# Autodesk Inventor assembly: Trappe Haute
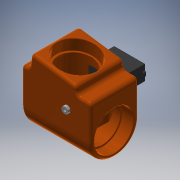
[picture p0: Inventor's stored thumbnail of the model, 180x180]
Saved by Autodesk Inventor 2016 SP1 (Build 200210100, 210)
## iProperties
Created: 2017-04-27
Part Number: Trappe Haute
Material: Générique
Document SubType Name: Assembly
Designer: dimercur
Author: dimercur
## Documents named in this file (6)
- D:\Users\dimercur\Documents\git\dev-gei\dev-gei2\Circuit-a-Bille\Trappe Haute.iam
- D:\Users\dimercur\Documents\git\dev-gei\dev-gei2\Circuit-a-Bille\Trappe Haute.ipt
- D:\Users\dimercur\Documents\git\dev-gei\dev-gei2\Circuit-a-Bille\Loquet Haut.ipt
- D:\Users\dimercur\Documents\git\dev-gei\dev-gei2\Circuit-a-Bille\Pieces importées\Futaba-s3004.ipt
- D:\Users\dimercur\Documents\Inventor\Content Center Files\R2016\fr-FR\NF E 25-130\NF E 25-130 - M5 x 10.ipt
- D:\Users\dimercur\Documents\Inventor\Content Center Files\R2016\fr-FR\ISO 7049 - F-H(2)\ISO 7049 - ST 3,5 x 9,5 - F - H.ipt
## Components (8 placed, 5 different names)
1. Trappe Haute:1 — Placage:6, Placage:7, Placage:10, Placage:11, Placage:12, Logement:1, Logement:2, Logement:3, Logement:4, Logement:5
2. Loquet Haut:1 — Placage:13, Placage:14
3. Futaba-s3004:1 — Placage:10, Placage:11, Placage:12, Placage:13, Placage:14
4. NF E 25-130 M5 x 10:1 — Logement:1
5. ISO 7049 - F-H ST 3,5 x 9,5 - F - H:1 — Logement:2
6. ISO 7049 - F-H ST 3,5 x 9,5 - F - H:2 — Logement:3
7. ISO 7049 - F-H ST 3,5 x 9,5 - F - H:3 — Logement:4
8. ISO 7049 - F-H ST 3,5 x 9,5 - F - H:4 — Logement:5
## Relationships (12: Mate 7, Insert 5)
- Placage:6 [Mate] (-30 mm): Trappe Haute:1
- Placage:7 [Mate] (-30 mm): Trappe Haute:1
- Placage:10 [Mate]: Trappe Haute:1 ↔ Futaba-s3004:1
- Placage:11 [Mate]: Trappe Haute:1 ↔ Futaba-s3004:1
- Placage:12 [Mate]: Trappe Haute:1 ↔ Futaba-s3004:1
- Placage:13 [Mate]: Loquet Haut:1 ↔ Futaba-s3004:1
- Placage:14 [Mate]: Loquet Haut:1 ↔ Futaba-s3004:1
- Logement:1 [Insert]: Trappe Haute:1 ↔ NF E 25-130 M5 x 10:1
- Logement:2 [Insert]: Trappe Haute:1 ↔ ISO 7049 - F-H ST 3,5 x 9,5 - F - H:1
- Logement:3 [Insert]: Trappe Haute:1 ↔ ISO 7049 - F-H ST 3,5 x 9,5 - F - H:2
- Logement:4 [Insert]: Trappe Haute:1 ↔ ISO 7049 - F-H ST 3,5 x 9,5 - F - H:3
- Logement:5 [Insert]: Trappe Haute:1 ↔ ISO 7049 - F-H ST 3,5 x 9,5 - F - H:4
